# Autodesk Inventor assembly: Assembly2
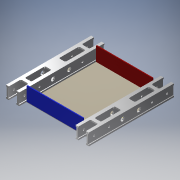
[picture p0: Inventor's stored thumbnail of the model, 180x180]
Saved by Autodesk Inventor 2017 (Build 210142000, 142)
## iProperties
Created: 2016-10-02
Part Number: Assembly2
Document SubType Name: Assembly
Designer: vslabsal
Author: vslabsal
## Documents named in this file (4)
- C:\Users\vslabsal\Documents\Assembly2.iam
- C:\Users\vslabsal\Documents\drive frame assembled.iam
- C:\Users\vslabsal\Documents\BasePlate-Short.ipt
- C:\Users\vslabsal\Documents\front back.ipt
## Components (5 placed, 3 different names)
1. drive frame assembled:1 [sub-assembly] — Rigid:2
2. drive frame assembled:2 [sub-assembly] — Rigid:1
3. BasePlate-Short:1 — Rigid:1, Rigid:2, Rigid:3, Rigid:4
4. front back:1 — Rigid:3
5. front back:2 — Rigid:4
## Relationships (4: WeldJoint 4)
- Rigid:1 [WeldJoint]: drive frame assembled:2 ↔ BasePlate-Short:1
- Rigid:2 [WeldJoint]: drive frame assembled:1 ↔ BasePlate-Short:1
- Rigid:3 [WeldJoint]: BasePlate-Short:1 ↔ front back:1
- Rigid:4 [WeldJoint]: BasePlate-Short:1 ↔ front back:2
